# Autodesk Inventor assembly: BBGW Case Assembly
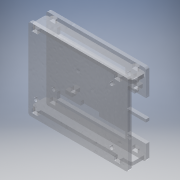
[picture p0: Inventor's stored thumbnail of the model, 180x180]
Saved by Autodesk Inventor 2016 (Build 200138000, 138)
## iProperties
Created: 2016-06-26
Part Number: BBGW Case Assembly
Document SubType Name: Assembly
Designer: Jacob
Author: Jacob
## Documents named in this file (5)
- H:\CAD\Hexapod\BBGW Case Assembly.iam
- H:\CAD\Hexapod\BBGW Case Bottom.ipt
- H:\CAD\Hexapod\BBGW Case Top.ipt
- H:\CAD\Hexapod\BBGW Case Side.ipt
- H:\CAD\Hexapod\BBGW Case Button.ipt
## Components (7 placed, 4 different names)
1. BBGW Case Bottom:1 — Mate:1, Mate:2, Mate:3, Mate:4, Mate:5, Mate:6
2. BBGW Case Top:1 — Mate:7, Mate:8, Mate:9, Mate:10, Mate:11, Mate:12, Mate:13, Mate:14, Mate:15, Mate:16, Mate:17, Mate:18
3. BBGW Case Side:1 — Mate:1, Mate:3, Mate:5, Mate:7, Mate:8, Mate:9
4. BBGW Case Side:2 — Mate:2, Mate:4, Mate:6
5. BBGW Case Button:1 — Mate:10, Mate:13, Mate:17
6. BBGW Case Button:2 — Mate:11, Mate:14, Mate:18
7. BBGW Case Button:3 — Mate:12, Mate:15, Mate:16
## Relationships (18: Mate 18)
- Mate:1: BBGW Case Bottom:1 ↔ BBGW Case Side:1
- Mate:2: BBGW Case Bottom:1 ↔ BBGW Case Side:2
- Mate:3: BBGW Case Bottom:1 ↔ BBGW Case Side:1
- Mate:4: BBGW Case Bottom:1 ↔ BBGW Case Side:2
- Mate:5: BBGW Case Bottom:1 ↔ BBGW Case Side:1
- Mate:6: BBGW Case Bottom:1 ↔ BBGW Case Side:2
- Mate:7: BBGW Case Top:1 ↔ BBGW Case Side:1
- Mate:8: BBGW Case Top:1 ↔ BBGW Case Side:1
- Mate:9: BBGW Case Top:1 ↔ BBGW Case Side:1
- Mate:10: BBGW Case Top:1 ↔ BBGW Case Button:1
- Mate:11: BBGW Case Top:1 ↔ BBGW Case Button:2
- Mate:12: BBGW Case Top:1 ↔ BBGW Case Button:3
- Mate:13: BBGW Case Top:1 ↔ BBGW Case Button:1
- Mate:14: BBGW Case Top:1 ↔ BBGW Case Button:2
- Mate:15: BBGW Case Top:1 ↔ BBGW Case Button:3
- Mate:16: BBGW Case Top:1 ↔ BBGW Case Button:3
- Mate:17: BBGW Case Top:1 ↔ BBGW Case Button:1
- Mate:18: BBGW Case Top:1 ↔ BBGW Case Button:2
